# Autodesk Inventor assembly: PIR sensor
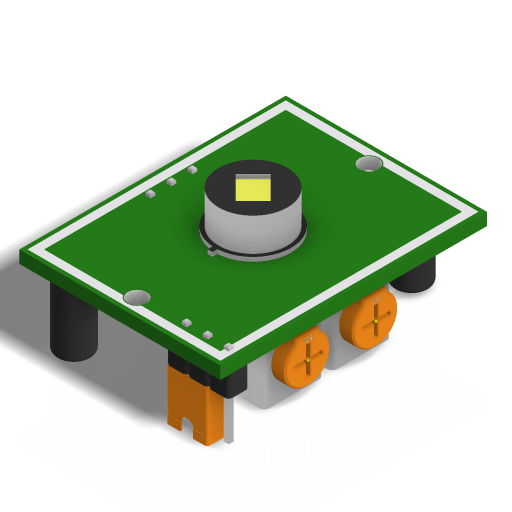
[picture p0: Inventor's stored thumbnail of the model, 512x512]
Saved by Autodesk Inventor 2024 (Build 280153000, 153)
## iProperties
Created: 2024-09-23
Part Number: PIR sensor
Document SubType Name: Assembly
Designer: Laith Al-Sadi
Author: Laith Al-Sadi
## Documents named in this file (11)
- D:\Sensors\PIR sensor.iam
- D:\Sensors\Board.ipt
- D:\Sensors\Fresnel lens.ipt
- D:\Sensors\BISS0001 Chip.ipt
- D:\Sensors\Pyroelectic sensor.ipt
- D:\Sensors\PIR pins.ipt
- D:\Sensors\Capacitor.ipt
- D:\Sensors\Time delay Adjust.ipt
- D:\Sensors\Sensitivity Adjust.ipt
- D:\Sensors\Retrigger Resetting Jumper.ipt
- D:\Sensors\3V DC Regulator.ipt
## Components (18 placed, 10 different names)
1. Board:1 — Mate:1, Flush:1, Mate:2, Flush:2, Mate:3, Flush:4, Angle:1, Mate:5, Flush:5, Mate:9, Mate:10, Flush:8, Mate:11, Mate:13, Tangent:1, Tangent:2, Mate:14, Tangent:3, Tangent:4, Tangent:5, Mate:16, Tangent:6, Tangent:7, Mate:17, Angle:2, Mate:18, Flush:10, Flush:11, Flush:14, Mate:22, Mate:23, Mate:24, Flush:15, Mate:28, Angle:4, Flush:16
2. Fresnel lens:1 — Mate:1, Flush:1, Mate:4, Flush:4
3. BISS0001 Chip:1 — Mate:2, Flush:2, Flush:8
4. Pyroelectic sensor:1 — Mate:3, Mate:4, Angle:1
5. PIR pins:1 — Mate:5, Flush:5, Mate:6, Mate:7, Mate:8, Flush:6, Flush:7
6. PIR pins:2 — Mate:8, Flush:6, Mate:9
7. PIR pins:3 — Mate:7, Flush:7, Mate:10
8. Capacitor:1 — Mate:11, Tangent:3, Tangent:4, Mate:15
9. Capacitor:2 — Mate:13, Tangent:2, Tangent:5
10. Capacitor:3 — Tangent:1, Mate:14, Mate:15, Tangent:8
11. Capacitor:4 — Mate:16, Tangent:6, Tangent:7
12. Time delay Adjust:1 — Mate:17, Angle:2, Angle:3, Flush:9, Flush:10, Mate:19, Flush:11
13. Sensitivity Adjust:1 — Mate:18, Angle:3, Flush:9, Mate:19
14. PIR pins:4 — Mate:23, Flush:15, Mate:25, Mate:26, Mate:27
15. PIR pins:5 — Flush:14, Mate:22
16. PIR pins:6 — Mate:24
17. Retrigger Resetting Jumper:1 — Mate:25, Mate:26, Mate:27
18. 3V DC Regulator:1 — Mate:28, Angle:4, Flush:16, Tangent:8
## Relationships (54: Mate 27, Flush 15, Tangent 8, Angle 4)
- Mate:1: Board:1 ↔ Fresnel lens:1
- Flush:1: Board:1 ↔ Fresnel lens:1
- Mate:2: Board:1 ↔ BISS0001 Chip:1
- Flush:2 (5 mm): Board:1 ↔ BISS0001 Chip:1
- Mate:3: Board:1 ↔ Pyroelectic sensor:1
- Mate:4: Fresnel lens:1 ↔ Pyroelectic sensor:1
- Flush:4 (5.1 mm): Board:1 ↔ Fresnel lens:1
- Angle:1 (45 deg): Board:1 ↔ Pyroelectic sensor:1
- Mate:5: Board:1 ↔ PIR pins:1
- Flush:5 (1 mm): Board:1 ↔ PIR pins:1
- Mate:6: PIR pins:1
- Mate:7: PIR pins:1 ↔ PIR pins:3
- Mate:8: PIR pins:1 ↔ PIR pins:2
- Flush:6: PIR pins:1 ↔ PIR pins:2
- Flush:7: PIR pins:1 ↔ PIR pins:3
- Mate:9: Board:1 ↔ PIR pins:2
- Mate:10: Board:1 ↔ PIR pins:3
- Flush:8 (6 mm): Board:1 ↔ BISS0001 Chip:1
- Mate:11: Board:1 ↔ Capacitor:1
- Mate:13: Board:1 ↔ Capacitor:2
- Tangent:1: Board:1 ↔ Capacitor:3
- Tangent:2: Board:1 ↔ Capacitor:2
- Mate:14: Board:1 ↔ Capacitor:3
- Tangent:3: Board:1 ↔ Capacitor:1
- Tangent:4 (5 mm): Board:1 ↔ Capacitor:1
- Tangent:5: Board:1 ↔ Capacitor:2
- Mate:15 (9 mm): Capacitor:1 ↔ Capacitor:3
- Mate:16: Board:1 ↔ Capacitor:4
- Tangent:6 (0.5 mm): Board:1 ↔ Capacitor:4
- Tangent:7 (2 mm): Board:1 ↔ Capacitor:4
- Mate:17: Board:1 ↔ Time delay Adjust:1
- Angle:2 (0 deg): Board:1 ↔ Time delay Adjust:1
- Mate:18: Board:1 ↔ Sensitivity Adjust:1
- Angle:3 (0 deg): Time delay Adjust:1 ↔ Sensitivity Adjust:1
- Flush:9: Time delay Adjust:1 ↔ Sensitivity Adjust:1
- Flush:10 (1 mm): Board:1 ↔ Time delay Adjust:1
- Mate:19 (1 mm): Time delay Adjust:1 ↔ Sensitivity Adjust:1
- Flush:11 (8 mm): Board:1 ↔ Time delay Adjust:1
- [Mate]: PIR pins:4 ↔ PIR pins:6
- [Mate]: PIR pins:4 ↔ PIR pins:5
- [Flush]: PIR pins:4 ↔ PIR pins:5
- [Flush]: PIR pins:4 ↔ PIR pins:6
- Flush:14: Board:1 ↔ PIR pins:5
- Mate:22: Board:1 ↔ PIR pins:5
- Mate:23: Board:1 ↔ PIR pins:4
- Mate:24: Board:1 ↔ PIR pins:6
- Flush:15 (1 mm): Board:1 ↔ PIR pins:4
- Mate:25: PIR pins:4 ↔ Retrigger Resetting Jumper:1
- Mate:26: PIR pins:4 ↔ Retrigger Resetting Jumper:1
- Mate:27: PIR pins:4 ↔ Retrigger Resetting Jumper:1
- Mate:28: Board:1 ↔ 3V DC Regulator:1
- Angle:4 (0 deg): Board:1 ↔ 3V DC Regulator:1
- Flush:16 (7 mm): Board:1 ↔ 3V DC Regulator:1
- Tangent:8: Capacitor:3 ↔ 3V DC Regulator:1
## Named parameters: d43_d14 = 0 mm, d44_d15 = 0 mm, d45_d16 = 0 mm, d46_d17 = 0 mm
